# Autodesk Inventor assembly: Swingarm2
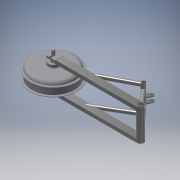
[picture p0: Inventor's stored thumbnail of the model, 180x180]
Saved by Autodesk Inventor 2018 (Build 220112000, 112)
## iProperties
Created: 2018-06-07
Part Number: Swingarm2
Document SubType Name: Assembly
Designer: eroldan
Author: eroldan
## Documents named in this file (3)
- C:\Users\eroldan\Desktop\3dprojects\OpenEmoto\Swingarm2\Swingarm2.iam
- C:\Users\eroldan\Desktop\3dprojects\OpenEmoto\OtherParts\HubMotor3KW.ipt
- C:\Users\eroldan\Desktop\3dprojects\OpenEmoto\Swingarm2\Swingarm2.ipt
## Components (2 placed, 2 different names)
1. HubMotor3KW:1 — Mate:1, Mate:2, Mate:3
2. Swingarm2:1 — Mate:1, Mate:2, Mate:3
## Relationships (3: Mate 3)
- Mate:1: HubMotor3KW:1 ↔ Swingarm2:1
- Mate:2: HubMotor3KW:1 ↔ Swingarm2:1
- Mate:3: HubMotor3KW:1 ↔ Swingarm2:1
